# Autodesk Inventor assembly: Assembly1タミヤダンパー 改
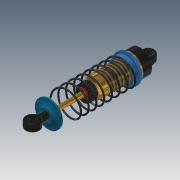
[picture p0: Inventor's stored thumbnail of the model, 180x180]
Saved by Autodesk Inventor 2020.1 (Build 241239000, 239)
## iProperties
Created: 2018-12-12
Part Number: Assembly1タミヤダンパー 改
Material: 一般
Document SubType Name: Assembly
Designer: 杉本　賢二郎
Mass: 28.9165 g
Surface Area: 73.8417 cm^2
Volume: 5.50756 cm^3
Density: 5.25032 g/cm^3
Author: 杉本　賢二郎
## Documents named in this file (5)
- G:\マイドライブ\青山穂高\ダンパー\Assembly1タミヤダンパー _フロント.iam
- G:\マイドライブ\青山穂高\ダンパー\Assembly2タミヤダンパー_フロント上.iam
- G:\マイドライブ\青山穂高\ダンパー\Assembly2タミヤダンパー_フロント下.iam
- G:\マイドライブ\青山穂高\ダンパー\タミヤダンパー部品9.ipt
- G:\マイドライブ\青山穂高\ダンパー\タミヤダンパー部品10_フロントバネ.ipt
## Components (4 placed, 4 different names)
1. Assembly2タミヤダンパー_フロント上:1 [sub-assembly] — 円柱状:2, フラッシュ:2
2. Assembly2タミヤダンパー_フロント下:1 [sub-assembly] — 円柱状:2, フラッシュ:2, 挿入:1
3. タミヤダンパー部品9:1 — 挿入:1
4. タミヤダンパー部品10_フロントバネ:1
## Relationships (3: CylindricalJoint 1, Flush 1, Insert 1)
- 円柱状:2 [CylindricalJoint]: Assembly2タミヤダンパー_フロント上:1 ↔ Assembly2タミヤダンパー_フロント下:1
- フラッシュ:2 [Flush]: Assembly2タミヤダンパー_フロント上:1 ↔ Assembly2タミヤダンパー_フロント下:1
- 挿入:1 [Insert]: Assembly2タミヤダンパー_フロント下:1 ↔ タミヤダンパー部品9:1
